# Autodesk Inventor assembly: 000-belt_liner_v2
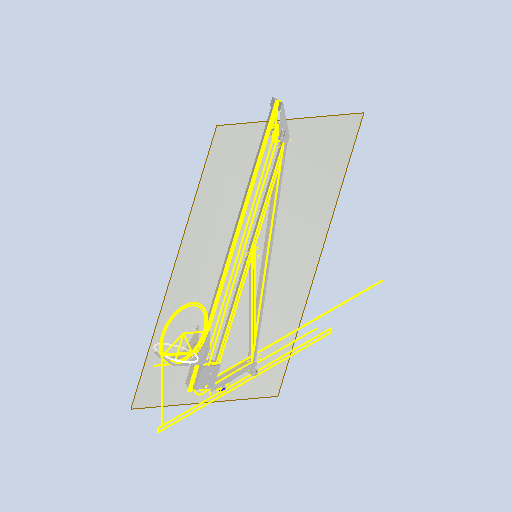
[picture p0: Inventor's stored thumbnail of the model, 512x512]
Saved by Autodesk Inventor 2025.2 (Build 292293000, 293)
## iProperties
Created: 2025-01-05
Part Number: 000-belt_liner_v2
Document SubType Name: Assembly
Designer: haruy
Author: haruy
## Documents named in this file (23)
- C:\Users\haruy\Documents\ロボコン\NHK2025\cad\nagahisa\belt_liner\000-belt_liner_v2.iam
- C:\Users\haruy\Documents\ロボコン\NHK2025\cad\nagahisa\belt_liner\belt_liner_v2_ASP_Base.ipt
- C:\Users\haruy\Documents\ロボコン\NHK2025\cad\nagahisa\belt_liner\belt_liner_v2_Plate_1.ipt
- C:\Users\haruy\Documents\ロボコン\NHK2025\cad\nagahisa\belt_liner\belt_liner_v2_Plate_2.ipt
- C:\Users\haruy\Documents\ロボコン\NHK2025\cad\nagahisa\belt_liner\belt_liner_v2_B_unit.ipt
- C:\Users\haruy\Documents\ロボコン\NHK2025\cad\nagahisa\belt_liner\belt_liner_v2_Plate_3.ipt
- C:\Users\haruy\Documents\ロボコン\NHK2025\cad\nagahisa\belt_liner\belt_liner_v2_Plate_4.ipt
- C:\Users\haruy\Documents\ロボコン\NHK2025\cad\nagahisa\belt_liner\belt_liner_v2_Plate_5.ipt
- C:\Users\haruy\Documents\ロボコン\NHK2025\cad\nagahisa\belt_liner\belt_liner_v2_Plate_6.ipt
- C:\Users\haruy\Documents\ロボコン\NHK2025\cad\nagahisa\belt_liner\belt_liner_v2_Plate_7.ipt
- C:\Users\haruy\Documents\ロボコン\NHK2025\cad\nagahisa\belt_liner\belt_liner_v2_Pom_r.ipt
- C:\Users\haruy\Documents\ロボコン\NHK2025\cad\nagahisa\belt_liner\belt_liner_v2_Plate_8.ipt
- C:\Users\haruy\Documents\ロボコン\NHK2025\cad\nagahisa\belt_liner\belt_liner_v2_Plate_9.ipt
- C:\Users\haruy\Documents\ロボコン\NHK2025\cad\nagahisa\belt_liner\belt_liner_v2_Plate_10.ipt
- C:\Users\haruy\Documents\ロボコン\NHK2025\cad\nagahisa\belt_liner\belt_liner_v2_Plate_11.ipt
- C:\Users\haruy\Documents\ロボコン\NHK2025\cad\nagahisa\belt_liner\belt_liner_v1_Plate_9.ipt
- C:\Users\haruy\Documents\ロボコン\NHK2025\cad\nagahisa\belt_liner\belt_liner_v2_Plate_12.ipt
- C:\Users\haruy\Documents\ロボコン\NHK2025\cad\nagahisa\belt_liner\C-SHFMQ20_b.ipt
- C:\Users\haruy\Documents\ロボコン\NHK2025\cad\nagahisa\belt_liner\roja-v1-3DP-rotate-spesa.ipt
- C:\Users\haruy\Documents\ロボコン\NHK2025\cad\nagahisa\belt_liner\roja-v1-Shaft-rotate.ipt
- C:\Users\haruy\Documents\ロボコン\NHK2025\cad\nagahisa\belt_liner\belt_liner_v2_Plate_13.ipt
- C:\Users\haruy\Documents\ロボコン\NHK2025\cad\nagahisa\belt_liner\belt_liner_v2_B_unit-2.ipt
- C:\Users\haruy\Documents\ロボコン\NHK2025\cad\nagahisa\belt_liner\belt_liner_v2_Plate_14.ipt
## Components (28 placed, 22 different names)
1. belt_liner_v2_ASP_Base:1 — 正接:1, 正接:2, 正接:3, 正接:4, 角度:1, 角度:2, 挿入:39, 挿入:40, 挿入:41, 挿入:42, 挿入:43, 挿入:44, 挿入:45, 挿入:46, 挿入:59, 挿入:60, 挿入:65, 挿入:66
2. belt_liner_v2_Plate_1:1 — 挿入:51, 挿入:52
3. belt_liner_v2_Plate_1:2 — 挿入:53, 挿入:54
4. belt_liner_v2_Plate_2:1 — 挿入:47, 挿入:48, 挿入:55, 挿入:56
5. belt_liner_v2_Plate_2:2 — 挿入:49, 挿入:50, 挿入:57, 挿入:58
6. belt_liner_v2_B_unit:1 — 挿入:21, 挿入:22, 挿入:23, 挿入:24, 正接:1, 正接:2, 正接:3, 正接:4
7. belt_liner_v2_Plate_3:1 — 挿入:21, 挿入:22, 角度:1, 角度:2
8. belt_liner_v2_Plate_4:1 — 挿入:23, 挿入:24, 挿入:25, 挿入:26, 挿入:27, 挿入:28, 挿入:29, 挿入:30, 挿入:31, 挿入:32
9. belt_liner_v2_Plate_5:1 — 挿入:25, 挿入:26
10. belt_liner_v2_Plate_5:2 — 挿入:27, 挿入:28
11. belt_liner_v2_Plate_6:1 — 挿入:29, 挿入:30, 挿入:33, 挿入:36
12. belt_liner_v2_Plate_6:2 — 挿入:31, 挿入:32, 挿入:34, 角度:3, 挿入:35
13. belt_liner_v2_Plate_7:1 — 挿入:35, 挿入:36, 角度:4, 挿入:37
14. belt_liner_v2_Plate_7:2 — 挿入:33, 挿入:34, 角度:3, 角度:4, 挿入:38
15. belt_liner_v2_Pom_r:1 — 挿入:37, 挿入:38
16. belt_liner_v2_Plate_8:1 — 挿入:45, 挿入:46, 挿入:51, 挿入:52, 挿入:53, 挿入:54
17. belt_liner_v2_Plate_9:1 — 挿入:43, 挿入:44
18. belt_liner_v2_Plate_10:1 — 挿入:41, 挿入:42
19. belt_liner_v2_Plate_11:1 — 挿入:39, 挿入:40, 挿入:47, 挿入:48, 挿入:49, 挿入:50
20. belt_liner_v1_Plate_9:1 — 挿入:57, 挿入:58
21. belt_liner_v1_Plate_9:2 — 挿入:55, 挿入:56
22. belt_liner_v2_Plate_12:1 — 挿入:59, 挿入:60, 挿入:61, 挿入:62
23. C-SHFMQ20_b:1 — 挿入:61, 挿入:62, 挿入:63, 挿入:64
24. roja-v1-3DP-rotate-spesa:1 — 挿入:63
25. roja-v1-Shaft-rotate:1 — 挿入:64
26. belt_liner_v2_Plate_13:1 — 挿入:65, 挿入:66, 挿入:67
27. belt_liner_v2_B_unit-2:1 — 挿入:67, 挿入:69, 挿入:70
28. belt_liner_v2_Plate_14:1 — 挿入:69, 挿入:70
## Relationships (57: Insert 49, Tangent 4, Angle 4)
- 挿入:21 [Insert]: belt_liner_v2_B_unit:1 ↔ belt_liner_v2_Plate_3:1
- 挿入:22 [Insert]: belt_liner_v2_B_unit:1 ↔ belt_liner_v2_Plate_3:1
- 挿入:23 [Insert]: belt_liner_v2_B_unit:1 ↔ belt_liner_v2_Plate_4:1
- 挿入:24 [Insert]: belt_liner_v2_B_unit:1 ↔ belt_liner_v2_Plate_4:1
- 正接:1 [Tangent]: belt_liner_v2_ASP_Base:1 ↔ belt_liner_v2_B_unit:1
- 正接:2 [Tangent]: belt_liner_v2_ASP_Base:1 ↔ belt_liner_v2_B_unit:1
- 正接:3 [Tangent]: belt_liner_v2_ASP_Base:1 ↔ belt_liner_v2_B_unit:1
- 正接:4 [Tangent]: belt_liner_v2_ASP_Base:1 ↔ belt_liner_v2_B_unit:1
- 角度:1 [Angle] (0 deg): belt_liner_v2_ASP_Base:1 ↔ belt_liner_v2_Plate_3:1
- 角度:2 [Angle] (0 deg): belt_liner_v2_ASP_Base:1 ↔ belt_liner_v2_Plate_3:1
- 挿入:25 [Insert]: belt_liner_v2_Plate_4:1 ↔ belt_liner_v2_Plate_5:1
- 挿入:26 [Insert]: belt_liner_v2_Plate_4:1 ↔ belt_liner_v2_Plate_5:1
- 挿入:27 [Insert]: belt_liner_v2_Plate_4:1 ↔ belt_liner_v2_Plate_5:2
- 挿入:28 [Insert]: belt_liner_v2_Plate_4:1 ↔ belt_liner_v2_Plate_5:2
- 挿入:29 [Insert]: belt_liner_v2_Plate_4:1 ↔ belt_liner_v2_Plate_6:1
- 挿入:30 [Insert]: belt_liner_v2_Plate_4:1 ↔ belt_liner_v2_Plate_6:1
- 挿入:31 [Insert]: belt_liner_v2_Plate_4:1 ↔ belt_liner_v2_Plate_6:2
- 挿入:32 [Insert]: belt_liner_v2_Plate_4:1 ↔ belt_liner_v2_Plate_6:2
- 挿入:33 [Insert]: belt_liner_v2_Plate_6:1 ↔ belt_liner_v2_Plate_7:2
- 挿入:34 [Insert]: belt_liner_v2_Plate_6:2 ↔ belt_liner_v2_Plate_7:2
- 角度:3 [Angle] (0 deg): belt_liner_v2_Plate_6:2 ↔ belt_liner_v2_Plate_7:2
- 挿入:35 [Insert]: belt_liner_v2_Plate_6:2 ↔ belt_liner_v2_Plate_7:1
- 挿入:36 [Insert]: belt_liner_v2_Plate_6:1 ↔ belt_liner_v2_Plate_7:1
- 角度:4 [Angle] (0 deg): belt_liner_v2_Plate_7:1 ↔ belt_liner_v2_Plate_7:2
- 挿入:37 [Insert]: belt_liner_v2_Plate_7:1 ↔ belt_liner_v2_Pom_r:1
- 挿入:38 [Insert]: belt_liner_v2_Plate_7:2 ↔ belt_liner_v2_Pom_r:1
- 挿入:39 [Insert]: belt_liner_v2_ASP_Base:1 ↔ belt_liner_v2_Plate_11:1
- 挿入:40 [Insert]: belt_liner_v2_ASP_Base:1 ↔ belt_liner_v2_Plate_11:1
- 挿入:41 [Insert]: belt_liner_v2_ASP_Base:1 ↔ belt_liner_v2_Plate_10:1
- 挿入:42 [Insert]: belt_liner_v2_ASP_Base:1 ↔ belt_liner_v2_Plate_10:1
- 挿入:43 [Insert]: belt_liner_v2_ASP_Base:1 ↔ belt_liner_v2_Plate_9:1
- 挿入:44 [Insert]: belt_liner_v2_ASP_Base:1 ↔ belt_liner_v2_Plate_9:1
- 挿入:45 [Insert]: belt_liner_v2_ASP_Base:1 ↔ belt_liner_v2_Plate_8:1
- 挿入:46 [Insert]: belt_liner_v2_ASP_Base:1 ↔ belt_liner_v2_Plate_8:1
- 挿入:47 [Insert]: belt_liner_v2_Plate_2:1 ↔ belt_liner_v2_Plate_11:1
- 挿入:48 [Insert]: belt_liner_v2_Plate_2:1 ↔ belt_liner_v2_Plate_11:1
- 挿入:49 [Insert]: belt_liner_v2_Plate_2:2 ↔ belt_liner_v2_Plate_11:1
- 挿入:50 [Insert]: belt_liner_v2_Plate_2:2 ↔ belt_liner_v2_Plate_11:1
- 挿入:51 [Insert]: belt_liner_v2_Plate_1:1 ↔ belt_liner_v2_Plate_8:1
- 挿入:52 [Insert]: belt_liner_v2_Plate_1:1 ↔ belt_liner_v2_Plate_8:1
- 挿入:53 [Insert]: belt_liner_v2_Plate_1:2 ↔ belt_liner_v2_Plate_8:1
- 挿入:54 [Insert]: belt_liner_v2_Plate_1:2 ↔ belt_liner_v2_Plate_8:1
- 挿入:55 [Insert]: belt_liner_v2_Plate_2:1 ↔ belt_liner_v1_Plate_9:2
- 挿入:56 [Insert]: belt_liner_v2_Plate_2:1 ↔ belt_liner_v1_Plate_9:2
- 挿入:57 [Insert]: belt_liner_v2_Plate_2:2 ↔ belt_liner_v1_Plate_9:1
- 挿入:58 [Insert]: belt_liner_v2_Plate_2:2 ↔ belt_liner_v1_Plate_9:1
- 挿入:59 [Insert]: belt_liner_v2_ASP_Base:1 ↔ belt_liner_v2_Plate_12:1
- 挿入:60 [Insert]: belt_liner_v2_ASP_Base:1 ↔ belt_liner_v2_Plate_12:1
- 挿入:61 [Insert]: belt_liner_v2_Plate_12:1 ↔ C-SHFMQ20_b:1
- 挿入:62 [Insert]: belt_liner_v2_Plate_12:1 ↔ C-SHFMQ20_b:1
- 挿入:63 [Insert]: C-SHFMQ20_b:1 ↔ roja-v1-3DP-rotate-spesa:1
- 挿入:64 [Insert]: C-SHFMQ20_b:1 ↔ roja-v1-Shaft-rotate:1
- 挿入:65 [Insert]: belt_liner_v2_ASP_Base:1 ↔ belt_liner_v2_Plate_13:1
- 挿入:66 [Insert]: belt_liner_v2_ASP_Base:1 ↔ belt_liner_v2_Plate_13:1
- 挿入:67 [Insert]: belt_liner_v2_Plate_13:1 ↔ belt_liner_v2_B_unit-2:1
- 挿入:69 [Insert]: belt_liner_v2_B_unit-2:1 ↔ belt_liner_v2_Plate_14:1
- 挿入:70 [Insert]: belt_liner_v2_B_unit-2:1 ↔ belt_liner_v2_Plate_14:1
